# Autodesk Inventor assembly: Z gantry
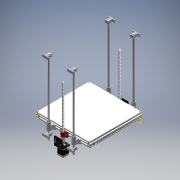
[picture p0: Inventor's stored thumbnail of the model, 180x180]
Saved by Autodesk Inventor 2018 (Build 220112000, 112)
## iProperties
Part Number: Z gantry
Material: Generisch
Document SubType Name: Assembly
Designer: Till
Author: Till
## Documents named in this file (20)
- C:\Users\Till\Dropbox\DIY\CoreBot\Z gantry.iam
- C:\Users\Till\Dropbox\DIY\CoreBot\steel rail 12mm.ipt
- C:\Users\Till\Dropbox\DIY\CoreBot\CAD Parts\SK12.ipt
- C:\Users\Till\Dropbox\DIY\CoreBot\CAD Parts\mutter_iso_4036_m4-st.ipt
- C:\Users\Till\Dropbox\DIY\CoreBot\CAD Parts\alu plate.ipt
- C:\Users\Till\Dropbox\DIY\CoreBot\CAD Parts\schraube_din_7991-m3x30-8_8.ipt
- C:\Users\Till\Dropbox\DIY\CoreBot\CAD Parts\375 - 8 (4 start) acme thread.ipt
- C:\Users\Till\Dropbox\DIY\CoreBot\CAD Parts\LeadScrew Nut 8mm x 2mmPitch.ipt
- C:\Users\Till\Dropbox\DIY\CoreBot\CAD Parts\5mm to 8mm flexible shaft coupler x.ipt
- C:\Users\Till\Dropbox\DIY\CoreBot\CAD Parts\Motor mount NEMA 17.ipt
- C:\Users\Till\Dropbox\DIY\CoreBot\CAD Parts\NEMA 17.ipt
- C:\Users\Till\Dropbox\DIY\CoreBot\CAD Parts\silicone heater.ipt
- C:\Users\Till\Dropbox\DIY\CAD\330mm.ipt
- C:\Users\Till\Dropbox\DIY\CAD\290mm.ipt
- C:\Users\Till\Dropbox\DIY\CoreBot\corner pieces + screw.iam
- C:\Users\Till\Dropbox\DIY\CoreBot\CAD Parts\screw_iso14580-m4x10-4_8.ipt
- C:\Users\Till\Dropbox\DIY\CoreBot\M3 x 10.ipt
- C:\Users\Till\Dropbox\DIY\CoreBot\Z flange.iam
- C:\Users\Till\Dropbox\DIY\CoreBot\Z nut mount.ipt
- C:\Users\Till\Dropbox\DIY\CoreBot\CAD Parts\item_0_0_654_96_5lsg25w4f0ghbh56jstw487ak.ipt
## Components (106 placed, 25 different names)
1. M3 x 10:26 — Fluchtend:194
2. M3 x 10:25 — Fluchtend:195, Passend:211
3. M3 x 10:24 — Fluchtend:196, Fluchtend:197, Passend:217
4. M3 x 10:23 — Fluchtend:199, Fluchtend:200, Passend:215
5. M3 x 10:22 — Fluchtend:201, Passend:214
6. M3 x 10:21 — Fluchtend:194, Passend:208
7. M3 x 10:20 — Fluchtend:198, Fluchtend:199, Passend:213
8. M3 x 10:19 — Fluchtend:195, Fluchtend:196, Passend:216
9. M3 x 10:18 — Fluchtend:200, Fluchtend:201, Passend:209, Passend:210
10. M3 x 10:17 — Fluchtend:197, Fluchtend:198, Passend:212
11. M3 x 10:8 — Fluchtend:149, Fluchtend:150, Passend:171
12. M3 x 10:7 — Fluchtend:149, Passend:170
13. M3 x 10:6 — Fluchtend:150, Fluchtend:151, Passend:169, Passend:172
14. M3 x 10:5 — Fluchtend:151, Passend:168
15. screw_iso14580-m4x10-4_8:2
16. screw_iso14580-m4x10-4_8:6
17. screw_iso14580-m4x10-4_8:7
18. screw_iso14580-m4x10-4_8:8
19. SK12 bottom right — Passend:12, Fluchtend:14, Fluchtend:5, Passend:115, Passend:129, Fluchtend:27, Fluchtend:28, Passend:214, Passend:215
20. steel rail 8mm right — Passend:1, Fluchtend:1, Passend:9, Fluchtend:3, Passend:12, Fluchtend:31, Passend:177
21. SK12 top right — Passend:9, Fluchtend:3, Fluchtend:4, Passend:127, Fluchtend:22, Fluchtend:23, Passend:209, Passend:210, Passend:212
22. NEMA 17:1 — Passend:116, Passend:117, Passend:118, Passend:119, Passend:161
23. Motor mount NEMA 17:1 — Fluchtend:20, Passend:114, Passend:115, Passend:116, Passend:117, Passend:118, Passend:133, Fluchtend:32, Fluchtend:33, Passend:168, Passend:169, Passend:170, Passend:171, Passend:172, Passend:208
24. 5mm to 8mm flexible shaft coupler x:1 — Passend:112, Passend:113, Passend:161
25. LeadScrew Nut 8mm x 2mmPitch:1 — Passend:111, Fluchtend:135, Passend:185, Passend:198, Passend:199, Passend:200, Passend:201, Passend:202
26. 375 - 8 (4 start) acme thread:1 — Passend:111, Passend:112, Passend:113, Passend:119, Passend:180
27. SK12 bottom left — Passend:10, Fluchtend:15, Fluchtend:14, Fluchtend:5, Fluchtend:20, Passend:114, Passend:130, Fluchtend:26, Fluchtend:29, Passend:216, Passend:217
28. SK12 top left — Passend:8, Fluchtend:2, Winkel:1, Fluchtend:4, Fluchtend:15, Passend:128, Fluchtend:24, Fluchtend:25, Passend:211, Passend:213
29. steel rail 12mm left — Passend:1, Fluchtend:1, Passend:8, Fluchtend:2, Passend:10, Fluchtend:30, Passend:176
30. M3 x 10:27 — Fluchtend:209, Passend:219, Passend:221
31. M3 x 10:28 — Fluchtend:206, Fluchtend:207, Passend:223
32. M3 x 10:29 — Fluchtend:205, Fluchtend:206, Passend:224
33. M3 x 10:30 — Fluchtend:208, Fluchtend:209, Passend:220
34. M3 x 10:31 — Fluchtend:207, Fluchtend:208, Passend:222
35. M3 x 10:32 — Fluchtend:202, Passend:218
36. M3 x 10:33 — Fluchtend:202
37. M3 x 10:34 — Fluchtend:203, Passend:225
38. M3 x 10:35 — Fluchtend:203, Fluchtend:204, Passend:227
39. M3 x 10:36 — Fluchtend:204, Fluchtend:205, Passend:226
40. M3 x 10:1 — Passend:164, Fluchtend:147
41. M3 x 10:2 — Passend:166, Fluchtend:146, Fluchtend:148
42. M3 x 10:3 — Passend:163, Fluchtend:147, Fluchtend:148
43. M3 x 10:4 — Passend:165, Fluchtend:146, Passend:167
44. screw_iso14580-m4x10-4_8:1
45. screw_iso14580-m4x10-4_8:3
46. screw_iso14580-m4x10-4_8:4
47. screw_iso14580-m4x10-4_8:5
48. SK12:5 — Passend:130, Fluchtend:26, Fluchtend:29, Passend:224, Passend:225
49. SK12:6 — Passend:128, Fluchtend:24, Fluchtend:25, Passend:131, Passend:222, Passend:223
50. SK12:7 — Passend:127, Fluchtend:22, Fluchtend:23, Passend:132, Passend:219, Passend:220, Passend:221
51. SK12:8 — Passend:129, Fluchtend:27, Fluchtend:28, Passend:226, Passend:227
52. steel rail 12mm:3 — Passend:131, Fluchtend:30, Passend:174
53. steel rail 12mm:4 — Passend:132, Fluchtend:31, Passend:175
54. 375 - 8 (4 start) acme thread:2 — Passend:181
55. LeadScrew Nut 8mm x 2mmPitch:2 — Fluchtend:135, Passend:183, Passend:184, Passend:203, Passend:204, Passend:205, Passend:206, Passend:207
56. 5mm to 8mm flexible shaft coupler x:2 — Passend:162
57. Motor mount NEMA 17:2 — Passend:133, Fluchtend:32, Fluchtend:33, Passend:163, Passend:164, Passend:165, Passend:166, Passend:167, Passend:218
58. NEMA 17:2 — Winkel:4, Passend:162
59. corner pieces + screw:1 [sub-assembly] — Passend:139, Passend:140, Fluchtend:144
60. corner pieces + screw:2 [sub-assembly] — Passend:141, Passend:142, Fluchtend:142
61. corner pieces + screw:3 [sub-assembly] — Passend:143, Passend:144, Fluchtend:145
62. corner pieces + screw:4 [sub-assembly] — Passend:137, Passend:138, Fluchtend:143
63. 330mm:1 — Passend:135, Fluchtend:139, Fluchtend:138, Passend:136, Fluchtend:140, Fluchtend:141, Passend:142, Passend:144, Winkel:3, Passend:173, Fluchtend:152
64. 330mm:3 — Passend:134, Fluchtend:136, Fluchtend:137, Passend:137, Passend:139, Winkel:2, Fluchtend:159
65. 290mm:1 — Passend:134, Fluchtend:136, Fluchtend:137, Passend:135, Fluchtend:139, Fluchtend:138, Passend:140, Passend:143, Fluchtend:144, Fluchtend:145, Winkel:6
66. 290mm:2 — Passend:136, Fluchtend:140, Fluchtend:141, Passend:138, Passend:141, Fluchtend:142, Fluchtend:143, Fluchtend:153, Passend:178, Winkel:5, Passend:179, Passend:182, Winkel:7
67. silicone heater:1 — Fluchtend:21, Fluchtend:34, Fluchtend:35
68. schraube_din_7991-m3x30-8_8:1 — Passend:80, Fluchtend:16, Passend:91, Passend:93, Passend:94
69. schraube_din_7991-m3x30-8_8:2 — Passend:83, Fluchtend:17, Passend:88, Passend:99, Passend:100
70. schraube_din_7991-m3x30-8_8:3 — Passend:81, Fluchtend:19, Passend:89, Passend:95, Passend:96
71. schraube_din_7991-m3x30-8_8:4 — Passend:82, Fluchtend:18, Passend:84, Passend:97, Passend:98
72. mutter_iso_4036_m4-st:9 — Passend:91
73. mutter_iso_4036_m4-st:10 — Passend:88
74. mutter_iso_4036_m4-st:11 — Passend:89
75. mutter_iso_4036_m4-st:12 — Passend:84
76. mutter_iso_4036_m4-st:13 — Passend:100, Passend:101
77. mutter_iso_4036_m4-st:14 — Passend:99
78. mutter_iso_4036_m4-st:15 — Passend:97
79. mutter_iso_4036_m4-st:16 — Passend:98, Passend:103
80. mutter_iso_4036_m4-st:17 — Passend:96
81. mutter_iso_4036_m4-st:18 — Passend:95, Passend:105
82. mutter_iso_4036_m4-st:19 — Passend:93
83. mutter_iso_4036_m4-st:20 — Passend:94, Passend:107
84. alu plate:1 — Passend:80, Fluchtend:16, Passend:81, Passend:82, Passend:83, Fluchtend:17, Fluchtend:18, Fluchtend:19, Passend:101, Passend:103, Passend:105, Passend:107, Fluchtend:21, Fluchtend:34, Fluchtend:35, Winkel:2, Winkel:3, Winkel:4, Passend:173, Fluchtend:152, Fluchtend:153
85. item_0_0_654_96_5lsg25w4f0ghbh56jstw487ak:8 — Fluchtend:191, Passend:203, Passend:204
86. item_0_0_654_96_5lsg25w4f0ghbh56jstw487ak:7 — Fluchtend:190, Passend:198, Passend:199
87. item_0_0_654_96_5lsg25w4f0ghbh56jstw487ak:6 — Fluchtend:189, Fluchtend:190, Passend:200
88. item_0_0_654_96_5lsg25w4f0ghbh56jstw487ak:5 — Fluchtend:188, Passend:201
89. item_0_0_654_96_5lsg25w4f0ghbh56jstw487ak:4 — Fluchtend:188, Fluchtend:189, Passend:202
90. item_0_0_654_96_5lsg25w4f0ghbh56jstw487ak:3 — Fluchtend:191, Fluchtend:192, Passend:206
91. item_0_0_654_96_5lsg25w4f0ghbh56jstw487ak:2 — Fluchtend:193, Passend:207
92. item_0_0_654_96_5lsg25w4f0ghbh56jstw487ak:1 — Fluchtend:192, Fluchtend:193, Passend:205
93. M3 x 10:16 — Fluchtend:187, Passend:193
94. M3 x 10:15 — Fluchtend:186, Passend:196
95. M3 x 10:14 — Fluchtend:187, Passend:192, Passend:194
96. M3 x 10:13 — Fluchtend:186, Passend:195, Passend:197
97. M3 x 10:12 — Fluchtend:184, Passend:186
98. M3 x 10:11 — Fluchtend:185, Passend:189, Passend:191
99. M3 x 10:10 — Fluchtend:185, Passend:190
100. M3 x 10:9 — Fluchtend:184, Passend:187, Passend:188
101. Z flange:1 [sub-assembly] — Fluchtend:156, Passend:175, Fluchtend:157, Passend:179, Fluchtend:159
102. Z flange:2 [sub-assembly] — Fluchtend:154, Fluchtend:155, Passend:177, Fluchtend:158
103. Z flange:3 [sub-assembly] — Fluchtend:154, Passend:176, Fluchtend:158
104. Z flange:4 [sub-assembly] — Fluchtend:155, Fluchtend:156, Passend:174, Fluchtend:157, Passend:178, Winkel:5
105. Z nut mount:1 — Passend:181, Fluchtend:183, Passend:182, Winkel:7, Passend:183, Passend:184, Passend:186, Passend:187, Passend:188, Passend:189, Passend:190, Passend:191
106. Z nut mount:2 — Passend:180, Fluchtend:183, Winkel:6, Passend:185, Passend:192, Passend:193, Passend:194, Passend:195, Passend:196, Passend:197
## Relationships (228: Mate 142, Flush 79, Angle 7)
- Passend:1 [Mate] (150 mm): steel rail 8mm right ↔ steel rail 12mm left
- Fluchtend:1 [Flush]: steel rail 8mm right ↔ steel rail 12mm left
- Passend:8 [Mate]: SK12 top left ↔ steel rail 12mm left
- Fluchtend:2 [Flush] (2 mm): SK12 top left ↔ steel rail 12mm left
- Winkel:1 [Angle] (0 deg): SK12 top left
- Passend:9 [Mate]: steel rail 8mm right ↔ SK12 top right
- Fluchtend:3 [Flush] (-2 mm): steel rail 8mm right ↔ SK12 top right
- Fluchtend:4 [Flush]: SK12 top right ↔ SK12 top left
- Passend:10 [Mate]: SK12 bottom left ↔ steel rail 12mm left
- Fluchtend:15 [Flush] (410 mm): SK12 bottom left ↔ SK12 top left
- Passend:12 [Mate]: SK12 bottom right ↔ steel rail 8mm right
- Fluchtend:14 [Flush]: SK12 bottom right ↔ SK12 bottom left
- Fluchtend:5 [Flush]: SK12 bottom right ↔ SK12 bottom left
- Passend:80 [Mate]: schraube_din_7991-m3x30-8_8:1 ↔ alu plate:1
- Fluchtend:16 [Flush]: schraube_din_7991-m3x30-8_8:1 ↔ alu plate:1
- Passend:81 [Mate]: schraube_din_7991-m3x30-8_8:3 ↔ alu plate:1
- Passend:82 [Mate]: schraube_din_7991-m3x30-8_8:4 ↔ alu plate:1
- Passend:83 [Mate]: schraube_din_7991-m3x30-8_8:2 ↔ alu plate:1
- Fluchtend:17 [Flush]: schraube_din_7991-m3x30-8_8:2 ↔ alu plate:1
- Fluchtend:18 [Flush]: schraube_din_7991-m3x30-8_8:4 ↔ alu plate:1
- Fluchtend:19 [Flush]: schraube_din_7991-m3x30-8_8:3 ↔ alu plate:1
- Passend:84 [Mate]: schraube_din_7991-m3x30-8_8:4 ↔ mutter_iso_4036_m4-st:12
- Passend:88 [Mate]: schraube_din_7991-m3x30-8_8:2 ↔ mutter_iso_4036_m4-st:10
- Passend:89 [Mate]: schraube_din_7991-m3x30-8_8:3 ↔ mutter_iso_4036_m4-st:11
- Passend:91 [Mate]: schraube_din_7991-m3x30-8_8:1 ↔ mutter_iso_4036_m4-st:9
- Passend:93 [Mate]: schraube_din_7991-m3x30-8_8:1 ↔ mutter_iso_4036_m4-st:19
- Passend:94 [Mate]: schraube_din_7991-m3x30-8_8:1 ↔ mutter_iso_4036_m4-st:20
- Passend:95 [Mate]: schraube_din_7991-m3x30-8_8:3 ↔ mutter_iso_4036_m4-st:18
- Passend:96 [Mate]: schraube_din_7991-m3x30-8_8:3 ↔ mutter_iso_4036_m4-st:17
- Passend:97 [Mate]: schraube_din_7991-m3x30-8_8:4 ↔ mutter_iso_4036_m4-st:15
- Passend:98 [Mate]: schraube_din_7991-m3x30-8_8:4 ↔ mutter_iso_4036_m4-st:16
- Passend:99 [Mate]: schraube_din_7991-m3x30-8_8:2 ↔ mutter_iso_4036_m4-st:14
- Passend:100 [Mate]: schraube_din_7991-m3x30-8_8:2 ↔ mutter_iso_4036_m4-st:13
- Passend:101 [Mate]: mutter_iso_4036_m4-st:13 ↔ alu plate:1
- Passend:103 [Mate]: mutter_iso_4036_m4-st:16 ↔ alu plate:1
- Passend:105 [Mate]: mutter_iso_4036_m4-st:18 ↔ alu plate:1
- Passend:107 [Mate]: mutter_iso_4036_m4-st:20 ↔ alu plate:1
- Passend:111 [Mate]: LeadScrew Nut 8mm x 2mmPitch:1 ↔ 375 - 8 (4 start) acme thread:1
- Passend:112 [Mate]: 5mm to 8mm flexible shaft coupler x:1 ↔ 375 - 8 (4 start) acme thread:1
- Passend:113 [Mate]: 5mm to 8mm flexible shaft coupler x:1 ↔ 375 - 8 (4 start) acme thread:1
- Fluchtend:20 [Flush]: Motor mount NEMA 17:1 ↔ SK12 bottom left
- Passend:114 [Mate] (-30 mm): Motor mount NEMA 17:1 ↔ SK12 bottom left
- Passend:115 [Mate] (65 mm): SK12 bottom right ↔ Motor mount NEMA 17:1
- Passend:116 [Mate]: NEMA 17:1 ↔ Motor mount NEMA 17:1
- Passend:117 [Mate]: NEMA 17:1 ↔ Motor mount NEMA 17:1
- Passend:118 [Mate]: NEMA 17:1 ↔ Motor mount NEMA 17:1
- Passend:119 [Mate]: NEMA 17:1 ↔ 375 - 8 (4 start) acme thread:1
- Fluchtend:21 [Flush]: silicone heater:1 ↔ alu plate:1
- [Mate]: 375 - 8 (4 start) acme thread:2 ↔ LeadScrew Nut 8mm x 2mmPitch:2
- [Mate]: 375 - 8 (4 start) acme thread:2 ↔ 5mm to 8mm flexible shaft coupler x:2
- [Mate]: 375 - 8 (4 start) acme thread:2 ↔ 5mm to 8mm flexible shaft coupler x:2
- [Mate]: Motor mount NEMA 17:2 ↔ NEMA 17:2
- [Mate]: Motor mount NEMA 17:2 ↔ NEMA 17:2
- [Mate]: Motor mount NEMA 17:2 ↔ NEMA 17:2
- [Mate]: 375 - 8 (4 start) acme thread:2 ↔ NEMA 17:2
- Passend:127 [Mate] (-400 mm): SK12 top right ↔ SK12:7
- Fluchtend:22 [Flush]: SK12 top right ↔ SK12:7
- Fluchtend:23 [Flush]: SK12 top right ↔ SK12:7
- Passend:128 [Mate] (-400 mm): SK12 top left ↔ SK12:6
- Fluchtend:24 [Flush]: SK12 top left ↔ SK12:6
- Fluchtend:25 [Flush]: SK12 top left ↔ SK12:6
- Passend:129 [Mate] (-400 mm): SK12 bottom right ↔ SK12:8
- Passend:130 [Mate] (-400 mm): SK12 bottom left ↔ SK12:5
- Fluchtend:26 [Flush]: SK12 bottom left ↔ SK12:5
- Fluchtend:27 [Flush]: SK12 bottom right ↔ SK12:8
- Fluchtend:28 [Flush]: SK12 bottom right ↔ SK12:8
- Fluchtend:29 [Flush]: SK12 bottom left ↔ SK12:5
- Passend:131 [Mate]: SK12:6 ↔ steel rail 12mm:3
- Passend:132 [Mate]: SK12:7 ↔ steel rail 12mm:4
- Fluchtend:30 [Flush]: steel rail 12mm left ↔ steel rail 12mm:3
- Fluchtend:31 [Flush]: steel rail 8mm right ↔ steel rail 12mm:4
- Passend:133 [Mate] (-400 mm): Motor mount NEMA 17:1 ↔ Motor mount NEMA 17:2
- Fluchtend:32 [Flush]: Motor mount NEMA 17:1 ↔ Motor mount NEMA 17:2
- Fluchtend:33 [Flush]: Motor mount NEMA 17:1 ↔ Motor mount NEMA 17:2
- Fluchtend:135 [Flush]: LeadScrew Nut 8mm x 2mmPitch:1 ↔ LeadScrew Nut 8mm x 2mmPitch:2
- Fluchtend:34 [Flush] (5 mm): silicone heater:1 ↔ alu plate:1
- Fluchtend:35 [Flush] (-5 mm): silicone heater:1 ↔ alu plate:1
- Passend:134 [Mate]: 330mm:3 ↔ 290mm:1
- Fluchtend:136 [Flush]: 330mm:3 ↔ 290mm:1
- Fluchtend:137 [Flush]: 330mm:3 ↔ 290mm:1
- Passend:135 [Mate]: 330mm:1 ↔ 290mm:1
- Fluchtend:139 [Flush]: 330mm:1 ↔ 290mm:1
- Fluchtend:138 [Flush]: 330mm:1 ↔ 290mm:1
- Passend:136 [Mate]: 330mm:1 ↔ 290mm:2
- Fluchtend:140 [Flush]: 330mm:1 ↔ 290mm:2
- Fluchtend:141 [Flush]: 330mm:1 ↔ 290mm:2
- Passend:137 [Mate]: corner pieces + screw:4 ↔ 330mm:3
- Passend:138 [Mate]: corner pieces + screw:4 ↔ 290mm:2
- Passend:139 [Mate]: corner pieces + screw:1 ↔ 330mm:3
- Passend:140 [Mate]: corner pieces + screw:1 ↔ 290mm:1
- Passend:141 [Mate]: corner pieces + screw:2 ↔ 290mm:2
- Passend:142 [Mate]: corner pieces + screw:2 ↔ 330mm:1
- Passend:143 [Mate]: corner pieces + screw:3 ↔ 290mm:1
- Passend:144 [Mate]: corner pieces + screw:3 ↔ 330mm:1
- Fluchtend:142 [Flush] (3.5 mm): corner pieces + screw:2 ↔ 290mm:2
- Fluchtend:143 [Flush] (3.5 mm): corner pieces + screw:4 ↔ 290mm:2
- Fluchtend:144 [Flush] (3.5 mm): corner pieces + screw:1 ↔ 290mm:1
- Fluchtend:145 [Flush] (3.5 mm): corner pieces + screw:3 ↔ 290mm:1
- [Mate]: screw_iso14580-m4x10-4_8:2 ↔ SK12 top left
- [Mate]: screw_iso14580-m4x10-4_8:7 ↔ SK12 top right
- [Mate]: screw_iso14580-m4x10-4_8:6 ↔ SK12 bottom left
- [Mate]: screw_iso14580-m4x10-4_8:8 ↔ SK12 bottom right
- [Mate]: screw_iso14580-m4x10-4_8:3 ↔ SK12:6
- [Mate]: screw_iso14580-m4x10-4_8:5 ↔ SK12:7
- [Mate]: screw_iso14580-m4x10-4_8:4 ↔ SK12:5
- [Mate]: screw_iso14580-m4x10-4_8:1 ↔ SK12:8
- [Mate]: screw_iso14580-m4x10-4_8:5 ↔ SK12:7
- [Mate]: screw_iso14580-m4x10-4_8:3 ↔ SK12:6
- [Mate]: screw_iso14580-m4x10-4_8:4 ↔ SK12:5
- [Mate]: screw_iso14580-m4x10-4_8:1 ↔ SK12:8
- [Mate]: screw_iso14580-m4x10-4_8:8 ↔ SK12 bottom right
- [Mate]: screw_iso14580-m4x10-4_8:6 ↔ SK12 bottom left
- [Mate]: screw_iso14580-m4x10-4_8:2 ↔ SK12 top left
- [Mate]: screw_iso14580-m4x10-4_8:7 ↔ SK12 top right
- Winkel:2 [Angle] (0 deg): 330mm:3 ↔ alu plate:1
- Winkel:3 [Angle] (0 deg): 330mm:1 ↔ alu plate:1
- Winkel:4 [Angle] (0 deg): NEMA 17:2 ↔ alu plate:1
- Passend:161 [Mate]: NEMA 17:1 ↔ 5mm to 8mm flexible shaft coupler x:1
- Passend:162 [Mate]: 5mm to 8mm flexible shaft coupler x:2 ↔ NEMA 17:2
- Passend:163 [Mate]: M3 x 10:3 ↔ Motor mount NEMA 17:2
- Passend:164 [Mate]: M3 x 10:1 ↔ Motor mount NEMA 17:2
- Passend:165 [Mate]: M3 x 10:4 ↔ Motor mount NEMA 17:2
- Passend:166 [Mate]: M3 x 10:2 ↔ Motor mount NEMA 17:2
- Fluchtend:146 [Flush]: M3 x 10:2 ↔ M3 x 10:4
- Fluchtend:147 [Flush]: M3 x 10:1 ↔ M3 x 10:3
- Fluchtend:148 [Flush]: M3 x 10:2 ↔ M3 x 10:3
- Passend:167 [Mate]: M3 x 10:4 ↔ Motor mount NEMA 17:2
- Fluchtend:149 [Flush]: M3 x 10:8 ↔ M3 x 10:7
- Fluchtend:150 [Flush]: M3 x 10:8 ↔ M3 x 10:6
- Fluchtend:151 [Flush]: M3 x 10:6 ↔ M3 x 10:5
- Passend:168 [Mate]: M3 x 10:5 ↔ Motor mount NEMA 17:1
- Passend:169 [Mate]: M3 x 10:6 ↔ Motor mount NEMA 17:1
- Passend:170 [Mate]: M3 x 10:7 ↔ Motor mount NEMA 17:1
- Passend:171 [Mate]: M3 x 10:8 ↔ Motor mount NEMA 17:1
- Passend:172 [Mate]: M3 x 10:6 ↔ Motor mount NEMA 17:1
- Passend:173 [Mate] (5 mm): 330mm:1 ↔ alu plate:1
- Fluchtend:152 [Flush] (5 mm): 330mm:1 ↔ alu plate:1
- Fluchtend:153 [Flush]: 290mm:2 ↔ alu plate:1
- Fluchtend:154 [Flush]: Z flange:2 ↔ Z flange:3
- Fluchtend:155 [Flush]: Z flange:2 ↔ Z flange:4
- Fluchtend:156 [Flush]: Z flange:1 ↔ Z flange:4
- Passend:174 [Mate]: steel rail 12mm:3 ↔ Z flange:4
- Passend:175 [Mate]: steel rail 12mm:4 ↔ Z flange:1
- Passend:176 [Mate]: steel rail 12mm left ↔ Z flange:3
- Passend:177 [Mate]: steel rail 8mm right ↔ Z flange:2
- Fluchtend:157 [Flush]: Z flange:1 ↔ Z flange:4
- Fluchtend:158 [Flush]: Z flange:2 ↔ Z flange:3
- Passend:178 [Mate]: 290mm:2 ↔ Z flange:4
- Winkel:5 [Angle] (180 deg): 290mm:2 ↔ Z flange:4
- Passend:179 [Mate]: 290mm:2 ↔ Z flange:1
- Fluchtend:159 [Flush] (55 mm): 330mm:3 ↔ Z flange:1
- Passend:180 [Mate]: 375 - 8 (4 start) acme thread:1 ↔ Z nut mount:2
- Passend:181 [Mate]: 375 - 8 (4 start) acme thread:2 ↔ Z nut mount:1
- Fluchtend:183 [Flush]: Z nut mount:1 ↔ Z nut mount:2
- Passend:182 [Mate]: 290mm:2 ↔ Z nut mount:1
- Winkel:6 [Angle] (180 deg): 290mm:1 ↔ Z nut mount:2
- Winkel:7 [Angle] (180 deg): 290mm:2 ↔ Z nut mount:1
- Passend:183 [Mate]: LeadScrew Nut 8mm x 2mmPitch:2 ↔ Z nut mount:1
- Passend:184 [Mate]: LeadScrew Nut 8mm x 2mmPitch:2 ↔ Z nut mount:1
- Passend:185 [Mate]: LeadScrew Nut 8mm x 2mmPitch:1 ↔ Z nut mount:2
- Fluchtend:184 [Flush]: M3 x 10:12 ↔ M3 x 10:9
- Fluchtend:185 [Flush]: M3 x 10:11 ↔ M3 x 10:10
- Passend:186 [Mate]: M3 x 10:12 ↔ Z nut mount:1
- Passend:187 [Mate]: M3 x 10:9 ↔ Z nut mount:1
- Passend:188 [Mate]: M3 x 10:9 ↔ Z nut mount:1
- Passend:189 [Mate]: M3 x 10:11 ↔ Z nut mount:1
- Passend:190 [Mate]: M3 x 10:10 ↔ Z nut mount:1
- Passend:191 [Mate]: M3 x 10:11 ↔ Z nut mount:1
- Fluchtend:186 [Flush]: M3 x 10:15 ↔ M3 x 10:13
- Fluchtend:187 [Flush]: M3 x 10:16 ↔ M3 x 10:14
- Passend:192 [Mate]: M3 x 10:14 ↔ Z nut mount:2
- Passend:193 [Mate]: M3 x 10:16 ↔ Z nut mount:2
- Passend:194 [Mate]: M3 x 10:14 ↔ Z nut mount:2
- Passend:195 [Mate]: M3 x 10:13 ↔ Z nut mount:2
- Passend:196 [Mate]: M3 x 10:15 ↔ Z nut mount:2
- Passend:197 [Mate]: M3 x 10:13 ↔ Z nut mount:2
- Fluchtend:188 [Flush]: item_0_0_654_96_5lsg25w4f0ghbh56jstw487ak:5 ↔ item_0_0_654_96_5lsg25w4f0ghbh56jstw487ak:4
- Fluchtend:189 [Flush]: item_0_0_654_96_5lsg25w4f0ghbh56jstw487ak:6 ↔ item_0_0_654_96_5lsg25w4f0ghbh56jstw487ak:4
- Fluchtend:190 [Flush]: item_0_0_654_96_5lsg25w4f0ghbh56jstw487ak:7 ↔ item_0_0_654_96_5lsg25w4f0ghbh56jstw487ak:6
- Passend:198 [Mate]: LeadScrew Nut 8mm x 2mmPitch:1 ↔ item_0_0_654_96_5lsg25w4f0ghbh56jstw487ak:7
- Passend:199 [Mate]: LeadScrew Nut 8mm x 2mmPitch:1 ↔ item_0_0_654_96_5lsg25w4f0ghbh56jstw487ak:7
- Passend:200 [Mate]: LeadScrew Nut 8mm x 2mmPitch:1 ↔ item_0_0_654_96_5lsg25w4f0ghbh56jstw487ak:6
- Passend:201 [Mate]: LeadScrew Nut 8mm x 2mmPitch:1 ↔ item_0_0_654_96_5lsg25w4f0ghbh56jstw487ak:5
- Passend:202 [Mate]: LeadScrew Nut 8mm x 2mmPitch:1 ↔ item_0_0_654_96_5lsg25w4f0ghbh56jstw487ak:4
- Fluchtend:191 [Flush]: item_0_0_654_96_5lsg25w4f0ghbh56jstw487ak:8 ↔ item_0_0_654_96_5lsg25w4f0ghbh56jstw487ak:3
- Fluchtend:192 [Flush]: item_0_0_654_96_5lsg25w4f0ghbh56jstw487ak:3 ↔ item_0_0_654_96_5lsg25w4f0ghbh56jstw487ak:1
- Fluchtend:193 [Flush]: item_0_0_654_96_5lsg25w4f0ghbh56jstw487ak:2 ↔ item_0_0_654_96_5lsg25w4f0ghbh56jstw487ak:1
- Passend:203 [Mate]: LeadScrew Nut 8mm x 2mmPitch:2 ↔ item_0_0_654_96_5lsg25w4f0ghbh56jstw487ak:8
- Passend:204 [Mate]: LeadScrew Nut 8mm x 2mmPitch:2 ↔ item_0_0_654_96_5lsg25w4f0ghbh56jstw487ak:8
- Passend:205 [Mate]: LeadScrew Nut 8mm x 2mmPitch:2 ↔ item_0_0_654_96_5lsg25w4f0ghbh56jstw487ak:1
- Passend:206 [Mate]: LeadScrew Nut 8mm x 2mmPitch:2 ↔ item_0_0_654_96_5lsg25w4f0ghbh56jstw487ak:3
- Passend:207 [Mate]: LeadScrew Nut 8mm x 2mmPitch:2 ↔ item_0_0_654_96_5lsg25w4f0ghbh56jstw487ak:2
- Fluchtend:194 [Flush]: M3 x 10:26 ↔ M3 x 10:21
- Passend:208 [Mate]: M3 x 10:21 ↔ Motor mount NEMA 17:1
- Fluchtend:195 [Flush]: M3 x 10:25 ↔ M3 x 10:19
- Fluchtend:196 [Flush]: M3 x 10:24 ↔ M3 x 10:19
- Fluchtend:197 [Flush]: M3 x 10:24 ↔ M3 x 10:17
- Fluchtend:198 [Flush]: M3 x 10:20 ↔ M3 x 10:17
- Fluchtend:199 [Flush]: M3 x 10:23 ↔ M3 x 10:20
- Fluchtend:200 [Flush]: M3 x 10:23 ↔ M3 x 10:18
- Fluchtend:201 [Flush]: M3 x 10:22 ↔ M3 x 10:18
- Passend:209 [Mate]: M3 x 10:18 ↔ SK12 top right
- Passend:210 [Mate]: M3 x 10:18 ↔ SK12 top right
- Passend:211 [Mate]: M3 x 10:25 ↔ SK12 top left
- Passend:212 [Mate]: M3 x 10:17 ↔ SK12 top right
- Passend:213 [Mate]: M3 x 10:20 ↔ SK12 top left
- Passend:214 [Mate]: M3 x 10:22 ↔ SK12 bottom right
- Passend:215 [Mate]: M3 x 10:23 ↔ SK12 bottom right
- Passend:216 [Mate]: M3 x 10:19 ↔ SK12 bottom left
- Passend:217 [Mate]: M3 x 10:24 ↔ SK12 bottom left
- Fluchtend:202 [Flush]: M3 x 10:32 ↔ M3 x 10:33
- Passend:218 [Mate]: M3 x 10:32 ↔ Motor mount NEMA 17:2
- Fluchtend:203 [Flush]: M3 x 10:34 ↔ M3 x 10:35
- Fluchtend:204 [Flush]: M3 x 10:35 ↔ M3 x 10:36
- Fluchtend:205 [Flush]: M3 x 10:29 ↔ M3 x 10:36
- Fluchtend:206 [Flush]: M3 x 10:28 ↔ M3 x 10:29
- Fluchtend:207 [Flush]: M3 x 10:28 ↔ M3 x 10:31
- Fluchtend:208 [Flush]: M3 x 10:30 ↔ M3 x 10:31
- Fluchtend:209 [Flush]: M3 x 10:27 ↔ M3 x 10:30
- Passend:219 [Mate]: M3 x 10:27 ↔ SK12:7
- Passend:220 [Mate]: M3 x 10:30 ↔ SK12:7
- Passend:221 [Mate]: M3 x 10:27 ↔ SK12:7
- Passend:222 [Mate]: M3 x 10:31 ↔ SK12:6
- Passend:223 [Mate]: M3 x 10:28 ↔ SK12:6
- Passend:224 [Mate]: M3 x 10:29 ↔ SK12:5
- Passend:225 [Mate]: M3 x 10:34 ↔ SK12:5
- Passend:226 [Mate]: M3 x 10:36 ↔ SK12:8
- Passend:227 [Mate]: M3 x 10:35 ↔ SK12:8
## Named parameters: d131_d120 = 0 mm, d132_d121 = 0 mm, d133_d122 = 0 mm, d134_d126 = 0 mm, d135_d127 = 0 mm, d136_d128 = 0 mm, d137_d129 = 0 mm
